# Autodesk Inventor assembly: spring_knob
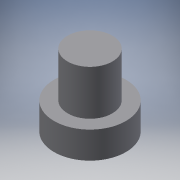
[picture p0: Inventor's stored thumbnail of the model, 180x180]
Saved by Autodesk Inventor 2017 (Build 210142000, 142)
## iProperties
Created: 2018-02-12
Part Number: spring_knob
Document SubType Name: Assembly
Designer: Nic
Author: Nic
## Documents named in this file (3)
- C:\Users\Nic\Documents\iDripper\spring_knob.iam
- C:\Users\Nic\Documents\iDripper\spring_hold_p1.ipt
- C:\Users\Nic\Documents\iDripper\spring_hold_p2.ipt
## Components (2 placed, 2 different names)
1. spring_hold_p1:1 — Insert:1
2. spring_hold_p2:1 — Insert:1
## Relationships (1: Insert 1)
- Insert:1: spring_hold_p1:1 ↔ spring_hold_p2:1
